# Autodesk Inventor assembly: leg_1_sim
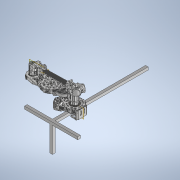
[picture p0: Inventor's stored thumbnail of the model, 180x180]
Saved by Autodesk Inventor 2020 (Build 240168000, 168)
## iProperties
Created: 2020-10-14
Part Number: leg_1_sim
Document SubType Name: Assembly
Designer: Shuang Peng
Author: Shuang Peng
## Documents named in this file (6)
- D:\projects-3\biped_gen1\hardware\leg_1_sim.iam
- D:\projects-3\biped_gen1\hardware\reducer_2.iam
- D:\projects-3\biped_gen1\hardware\reducer_leg.iam
- D:\projects-3\biped_gen1\hardware\sub_leg_1_lit.iam
- D:\projects-3\biped_gen1\hardware\leg_sim_stand.ipt
- D:\projects-3\biped_gen1\hardware\joint_ref.ipt
## Components (6 placed, 5 different names)
1. leg_sim_stand:1 — Mate:1, Mate:2
2. reducer_2:1 [sub-assembly] — Mate:1, Mate:2, Insert:1, Mate:3
3. reducer_leg:1 [sub-assembly] — Insert:1, Insert:2, Insert:4
4. sub_leg_1_lit:1 [sub-assembly] — Insert:2, Mate:3, Insert:3
5. joint_ref:1 — Insert:3
6. joint_ref:2 — Insert:4
## Relationships (7: Insert 4, Mate 3)
- Mate:1 (10 mm): leg_sim_stand:1 ↔ reducer_2:1
- Mate:2 (20 mm): leg_sim_stand:1 ↔ reducer_2:1
- Insert:1: reducer_2:1 ↔ reducer_leg:1
- Insert:2: reducer_leg:1 ↔ sub_leg_1_lit:1
- Mate:3: reducer_2:1 ↔ sub_leg_1_lit:1
- Insert:3: sub_leg_1_lit:1 ↔ joint_ref:1
- Insert:4: reducer_leg:1 ↔ joint_ref:2
